# Autodesk Inventor assembly: PCB_board
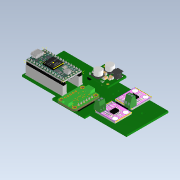
[picture p0: Inventor's stored thumbnail of the model, 180x180]
Saved by Autodesk Inventor 2020 (Build 240168000, 168)
## iProperties
Company: Open CASCADE
Created: 2021-03-04
Part Number: PCB_board
Description: Open CASCADE Model
Document SubType Name: Assembly
Designer: DELL
Authority: Unknown
Sending System: Open CASCADE 6.8
Preprocessor: Open CASCADE STEP processor 6.8
Title: Open CASCADE Shape Model
Author: Author
## Documents named in this file (8)
- F:\SoftRobot2.0\FlexipodHardware2.0\FlexipodHardware\Flexipod2.0\PCB\PCB_board.iam
- F:\SoftRobot2.0\FlexipodHardware2.0\FlexipodHardware\Flexipod2.0\PCB\Board.iam
- F:\SoftRobot2.0\FlexipodHardware2.0\FlexipodHardware\Flexipod2.0\PCB\connector_for_teensy.iam
- F:\SoftRobot2.0\FlexipodHardware2.0\FlexipodHardware\Flexipod2.0\PCB\teensy_4.0\teensy_4.0.iam
- F:\SoftRobot2.0\FlexipodHardware2.0\FlexipodHardware\Flexipod2.0\PCB\CAN_transceiver\CAN_transceiver_with_pins.iam
- F:\SoftRobot2.0\FlexipodHardware2.0\FlexipodHardware\Flexipod2.0\PCB\Adafruit-LSM6DSOX-LIS3MDL-PCB\Adafruit_LIS3MDL_LSM6DSOX.iam
- F:\SoftRobot2.0\FlexipodHardware2.0\FlexipodHardware\Flexipod2.0\PCB\Voltage_Regulator\d24v50f5-step-down-voltage-regulator.ipt
- F:\SoftRobot2.0\FlexipodHardware2.0\FlexipodHardware\Flexipod2.0\PCB\pins.ipt
## Components (17 placed, 7 different names)
1. Board_18 [sub-assembly] — Mate:1, Flush:1, Mate:2, Mate:6, Mate:8, Mate:9, Mate:17, Mate:18, Mate:26, Mate:29, Mate:30, Mate:31, Mate:32, Mate:34, Mate:35
2. connector_for_teensy_24 [sub-assembly] — Mate:1, Flush:1, Flush:2, Mate:3
3. teensy_4.0:1 [sub-assembly] — Flush:2, Mate:2, Mate:3
4. CAN_transceiver_with_pins:1 [sub-assembly] — Mate:8, Mate:30, Mate:31
5. CAN_transceiver_with_pins:2 [sub-assembly] — Mate:6, Mate:9, Mate:32
6. Adafruit_LIS3MDL_LSM6DSOX:1 [sub-assembly] — Mate:25, Mate:27, Mate:33, Mate:35
7. d24v50f5-step-down-voltage-regulator:1 — Mate:15, Mate:16, Mate:28
8. pins:1 — Flush:3, Flush:6, Mate:14, Mate:15, Mate:16, Mate:17
9. pins:2 — Flush:3, Flush:4, Flush:6, Flush:7, Mate:13, Mate:14
10. pins:3 — Flush:4, Flush:5, Flush:7, Flush:8, Mate:12, Mate:13
11. pins:4 — Flush:5, Flush:8, Mate:12, Mate:18, Mate:28, Mate:29
12. pins:5 — Mate:33, Mate:34
13. pins:6
14. pins:7
15. pins:8 — Mate:23, Flush:17, Flush:18
16. pins:9 — Mate:23, Flush:17, Flush:18
17. pins:10 — Mate:25, Mate:26, Mate:27
## Relationships (47: Mate 29, Flush 18)
- Mate:1: Board_18 ↔ connector_for_teensy_24
- Flush:1 (2 mm): Board_18 ↔ connector_for_teensy_24
- Flush:2: connector_for_teensy_24 ↔ teensy_4.0:1
- Mate:2: Board_18 ↔ teensy_4.0:1
- Mate:3: connector_for_teensy_24 ↔ teensy_4.0:1
- Mate:6: Board_18 ↔ CAN_transceiver_with_pins:2
- Mate:8: Board_18 ↔ CAN_transceiver_with_pins:1
- Mate:9: Board_18 ↔ CAN_transceiver_with_pins:2
- Flush:3: pins:1 ↔ pins:2
- Flush:4: pins:2 ↔ pins:3
- Flush:5: pins:3 ↔ pins:4
- Flush:6: pins:1 ↔ pins:2
- Flush:7: pins:2 ↔ pins:3
- Flush:8: pins:3 ↔ pins:4
- Mate:12: pins:3 ↔ pins:4
- Mate:13: pins:2 ↔ pins:3
- Mate:14: pins:1 ↔ pins:2
- Mate:15: d24v50f5-step-down-voltage-regulator:1 ↔ pins:1
- Mate:16: d24v50f5-step-down-voltage-regulator:1 ↔ pins:1
- Mate:17: Board_18 ↔ pins:1
- Mate:18: Board_18 ↔ pins:4
- [Flush]: pins:5 ↔ pins:6
- [Flush]: pins:6 ↔ pins:7
- [Flush]: pins:7 ↔ pins:8
- [Flush]: pins:5 ↔ pins:6
- [Flush]: pins:6 ↔ pins:7
- [Flush]: pins:7 ↔ pins:8
- [Mate]: pins:7 ↔ pins:8
- [Mate]: pins:6 ↔ pins:7
- [Mate]: pins:5 ↔ pins:6
- [Flush]: pins:9 ↔ pins:10
- [Flush]: pins:9 ↔ pins:10
- [Mate]: pins:9 ↔ pins:10
- Mate:23: pins:8 ↔ pins:9
- Flush:17: pins:8 ↔ pins:9
- Flush:18: pins:8 ↔ pins:9
- Mate:25: Adafruit_LIS3MDL_LSM6DSOX:1 ↔ pins:10
- Mate:26: Board_18 ↔ pins:10
- Mate:27: Adafruit_LIS3MDL_LSM6DSOX:1 ↔ pins:10
- Mate:28: d24v50f5-step-down-voltage-regulator:1 ↔ pins:4
- Mate:29: Board_18 ↔ pins:4
- Mate:30: Board_18 ↔ CAN_transceiver_with_pins:1
- Mate:31: Board_18 ↔ CAN_transceiver_with_pins:1
- Mate:32: Board_18 ↔ CAN_transceiver_with_pins:2
- Mate:33: Adafruit_LIS3MDL_LSM6DSOX:1 ↔ pins:5
- Mate:34: Board_18 ↔ pins:5
- Mate:35: Board_18 ↔ Adafruit_LIS3MDL_LSM6DSOX:1
## Named parameters: d26_d13 = 0 mm, d27_d14 = 0 mm, d28_d15 = 0 mm, d29_d16 = 0 mm, d30_d17 = 0 mm, d31_d18 = 0 mm, d32_d19 = 0 mm, d33_d20 = 0 mm, d34_d21 = 0 mm, d35_d28_d15 = 0 mm, d36_d31_d18 = 0 mm, d37_d32_d19 = 0 mm
